# Autodesk Inventor assembly: PZT Assembly Modified
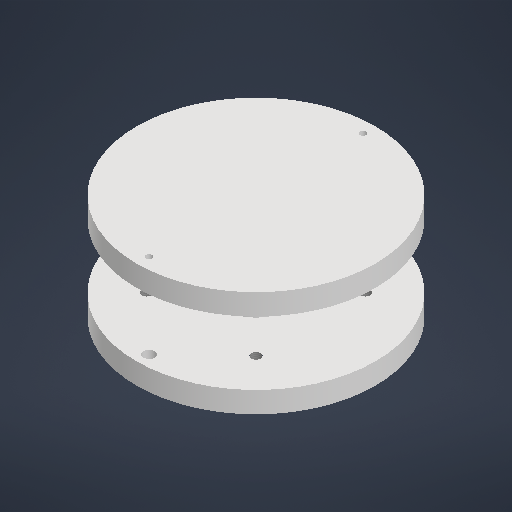
[picture p0: Inventor's stored thumbnail of the model, 512x512]
Saved by Autodesk Inventor 2025 (Build 290162000, 162)
## iProperties
Created: 2024-07-03
Part Number: PZT Assembly Modified
Document SubType Name: Assembly
Designer: mayhe
Author: mayhe
## Documents named in this file (4)
- C:\Users\mayhe\OneDrive\Documents\GitHub\In-situ-monitoring-of-powder-bed-fusion-additive-manufacturing\system_development\Orichalcum\v0.2\Hardware_design\pzt-parts\PZT Assembly Modified.iam
- C:\Users\mayhe\OneDrive\Documents\GitHub\In-situ-monitoring-of-powder-bed-fusion-additive-manufacturing\system_development\Orichalcum\v0.2\Hardware_design\pzt-parts\Modified Substrate Plate Bottom.ipt
- C:\Users\mayhe\OneDrive\Documents\GitHub\In-situ-monitoring-of-powder-bed-fusion-additive-manufacturing\system_development\Orichalcum\v0.2\Hardware_design\pzt-parts\Modified Substrate Plate Top.ipt
- C:\Users\mayhe\OneDrive\Documents\GitHub\In-situ-monitoring-of-powder-bed-fusion-additive-manufacturing\system_development\Orichalcum\v0.2\Hardware_design\pzt-parts\shaker cut.ipt
## Components (3 placed, 3 different names)
1. Modified Substrate Plate Top:1 — Rotational:1
2. shaker cut:1 — Rotational:1, Rotational:2
3. Modified Substrate Plate Bottom:1 — Rotational:2
## Relationships (2: RevoluteJoint 2)
- Rotational:1 [RevoluteJoint]: Modified Substrate Plate Top:1 ↔ shaker cut:1
- Rotational:2 [RevoluteJoint]: shaker cut:1 ↔ Modified Substrate Plate Bottom:1
